# Autodesk Inventor assembly: ASM0002_ASM
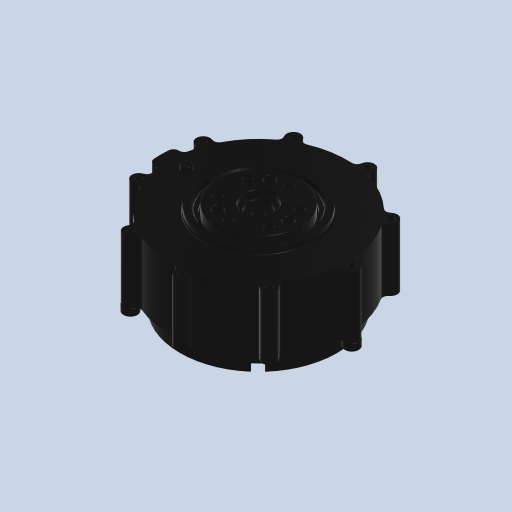
[picture p0: Inventor's stored thumbnail of the model, 512x512]
Saved by Autodesk Inventor 2023 (Build 270158000, 158)
## iProperties
Created: 2023-09-07
Part Number: ASM0002_ASM
Document SubType Name: Assembly
Designer: kiyo
Mass: 113.975 g
Surface Area: 460.475 cm^2
Volume: 112.555 cm^3
Density: 1.01262 g/cm^3
Sending System: CREO PARAMETRIC BY PTC INC, 2017260
Preprocessor: CREO PARAMETRIC BY PTC INC, 2017260
Title: ASM0002_ASM
Author: liu
Revision Number: 1LAST_VERSION
## Documents named in this file (3)
- D:\GitHub\inventor\OfficeRobot\ReadyMade\CyberGear\CyberGearmotor.iam
- D:\GitHub\inventor\OfficeRobot\ReadyMade\CyberGear\ASM0002_ASM_1_ASM.iam
- D:\GitHub\inventor\OfficeRobot\ReadyMade\CyberGear\0411-2_4_1_3_1.ipt
## Components (2 placed, 2 different names)
1. 20 [sub-assembly] — 挿入:1, 挿入:2, 角度:1, 角度:2
2. 21 — 挿入:1, 挿入:2
## Relationships (4: Insert 2, Angle 2)
- 挿入:1 [Insert]: 20 ↔ 21
- 挿入:2 [Insert]: 20 ↔ 21
- 角度:1 [Angle] (0 deg): 20
- 角度:2 [Angle] (0 deg): 20
